# Autodesk Inventor assembly: Shooter Assembly
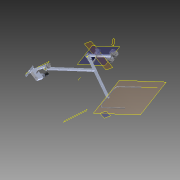
[picture p0: Inventor's stored thumbnail of the model, 180x180]
Saved by Autodesk Inventor 2014 (Build 180170000, 170)
## iProperties
Created: 2014-01-05
Part Number: Shooter Assembly
Document SubType Name: Assembly
Designer: Andrew Toennies
Mass: 1582.87 g
Surface Area: 6510.69 cm^2
Volume: 621.462 cm^3
Density: 2.54701 g/cm^3
Author: Andrew Toennies
## Documents named in this file (30)
- C:\Users\Andrew Toennies\Documents\GitHub\2014buildCAD\Shooter\Shooter Assembly.iam
- C:\Users\Andrew Toennies\Documents\GitHub\2014buildCAD\Shooter\Vex Pro 1x1 rectangular tubing 12 in length.ipt
- C:\Users\Andrew Toennies\Documents\GitHub\2014buildCAD\Shooter\Vex Pro End Bearing Mount.ipt
- C:\Users\Andrew Toennies\Documents\GitHub\2014buildCAD\Shooter\Vex Pro 1x1 rectangular tubing 27 in length.ipt
- C:\Users\Andrew Toennies\Documents\GitHub\2014buildCAD\Shooter\Vex Pro 1x1 rectangular tubing 24 in length.ipt
- C:\Users\Andrew Toennies\Documents\GitHub\2014buildCAD\Shooter\Vex Pro T gusset.ipt
- C:\Users\Andrew Toennies\Documents\GitHub\2014buildCAD\Shooter\Vex Pro Corner Gusset.ipt
- C:\Users\Andrew Toennies\Documents\GitHub\2014buildCAD\Shooter\Vex Pro 1x1 rectangular tubing 13 in length.ipt
- C:\Users\Andrew Toennies\Documents\GitHub\2014buildCAD\Shooter\Vex Pro Side Bearing Gusset.ipt
- C:\Users\Andrew Toennies\Documents\GitHub\2014buildCAD\Shooter\Bearing ID 0.500 Hex OD 1.125.ipt
- C:\Users\Andrew Toennies\Documents\GitHub\2014buildCAD\Shooter\Axle 0.500 Hex 5 in length.ipt
- C:\Users\Andrew Toennies\Documents\GitHub\2014buildCAD\Shooter\Spacer.ipt
- C:\Users\Andrew Toennies\Documents\GitHub\2014buildCAD\Shooter\Bearing ID 0.375 OD 1.125.ipt
- C:\Users\Andrew Toennies\Documents\GitHub\2014buildCAD\Shooter\Axle 0.375 3 in length.ipt
- C:\Users\Andrew Toennies\Documents\GitHub\2014buildCAD\Shooter\Vex Pro 30 tooth 9mm timing belt pulley.ipt
- C:\Users\Andrew Toennies\Documents\GitHub\2014buildCAD\Shooter\Vex Pro VersaHub 0.500 Hex.ipt
- C:\Users\Andrew Toennies\Documents\GitHub\2014buildCAD\Shooter\armbackspacer.ipt
- C:\Users\Andrew Toennies\Documents\GitHub\2014buildCAD\Shooter\Axle 0.500 Hex 3 in length.ipt
- C:\Users\Andrew Toennies\Documents\GitHub\2014buildCAD\Shooter\Worm-Drive-Gearbox-16to1.iam
- C:\Users\Andrew Toennies\Documents\GitHub\2014buildCAD\Shooter\Vex Pro 32 tooth 15 mm timing belt pulley.ipt
- C:\Users\Andrew Toennies\Documents\GitHub\2014buildCAD\Shooter\Vex Pro Traction 1 in wide 4 in dia wheel.iam
- C:\Users\Andrew Toennies\Documents\GitHub\2014buildCAD\Shooter\Aluminum Tube Bent 0.500 OD 0.436 ID.ipt
- C:\Users\Andrew Toennies\Documents\GitHub\2014buildCAD\Shooter\Bag Motor with VersaPlanetary 10 to 1 Reduction.iam
- C:\Users\Andrew Toennies\Documents\GitHub\2014buildCAD\Shooter\Vex Pro 18 tooth timing belt pulley.ipt
- C:\Users\Andrew Toennies\Documents\GitHub\2014buildCAD\Shooter\Vex Pro VersaPlanetary Face Mount.ipt
- C:\Users\Andrew Toennies\Documents\GitHub\2014buildCAD\Shooter\Pneumatic Cylinder Retracted (McMaster Part #6498K602).ipt
- C:\Users\Andrew Toennies\Documents\GitHub\2014buildCAD\Shooter\Foot Bracket Mount (McMaster Part #6498K710).ipt
- C:\Users\Andrew Toennies\Documents\GitHub\2014buildCAD\Shooter\Rod End (McMaster Part #6498K592).ipt
- C:\Users\Andrew Toennies\Documents\GitHub\2014buildCAD\Shooter\Spacer2.ipt
- C:\Users\Andrew Toennies\Documents\GitHub\2014buildCAD\Shooter\Bracket.ipt
## Components (46 placed, 29 different names)
1. Vex Pro 1x1 rectangular tubing 12 in length:1 — Flush:1, Insert:9, Insert:10, Insert:11, Insert:12, Flush:4, Mate:23, Mate:24, Mate:25, Mate:26, Mate:27, Mate:28, Mate:43, Mate:49, Mate:50, Angle:1
2. Vex Pro 1x1 rectangular tubing 27 in length:1 — Flush:1, Insert:5, Insert:6, Insert:7, Insert:8, Flush:2, Mate:2, Mate:33, Mate:34
3. Vex Pro 1x1 rectangular tubing 24 in length:1 — Flush:2, Mate:2, Flush:3, Mate:6, Flush:9, Mate:53, Mate:54, Angle:1, Flush:17, Angle:2, Flush:22, Flush:23, Mate:64, Mate:65, Flush:24, Insert:57, Insert:58
4. Vex Pro T gusset:1 — Insert:5, Insert:6, Mate:6
5. Vex Pro T gusset:2 — Insert:7, Insert:8
6. Vex Pro Corner Gusset:1 — Insert:9, Insert:10, Flush:6
7. Vex Pro Corner Gusset:2 — Insert:11, Insert:12
8. Vex Pro End Bearing Mount:3 — Insert:35, Insert:47, Insert:48, Angle:3
9. Vex Pro End Bearing Mount:4 — Insert:36, Insert:49, Insert:50
10. Vex Pro 1x1 rectangular tubing 13 in length:1 — Flush:3, Insert:21, Insert:22, Insert:23, Insert:24, Flush:8, Mate:51, Angle:2, Flush:19, Flush:20, Flush:21, Mate:63, Flush:25, Tangent:1, Insert:59, Insert:60, Insert:61, Insert:62
11. Vex Pro End Bearing Mount:5 — Insert:21, Insert:22, Insert:25
12. Vex Pro End Bearing Mount:6 — Insert:23, Insert:24, Insert:26
13. Bearing ID 0.500 Hex OD 1.125:1 — Insert:26, Flush:7, Mate:7, Mate:8
14. Bearing ID 0.500 Hex OD 1.125:2 — Insert:25, Flush:7, Mate:10, Mate:16
15. Axle 0.500 Hex 5 in length:1 — Mate:7, Mate:8, Flush:8, Flush:10, Flush:11, Mate:14, Mate:15, Mate:18, Mate:19, Mate:21, Mate:22, Flush:12, Flush:16
16. Spacer:1 — Insert:47, Insert:48, Mate:65, Flush:24
17. Spacer:2 — Insert:49, Insert:50, Flush:22, Flush:23, Mate:64
18. Bearing ID 0.375 OD 1.125:1 — Insert:35, Mate:9
19. Bearing ID 0.375 OD 1.125:2 — Insert:36, Mate:66
20. Axle 0.375 3 in length:1 — Mate:9, Flush:9, Mate:13, Mate:51, Mate:66
21. Vex Pro 30 tooth 9mm timing belt pulley:1 — Mate:14, Mate:15, Mate:16, Flush:18
22. Vex Pro VersaHub 0.500 Hex:1 — Mate:17, Mate:18, Mate:19, Flush:16, Insert:51
23. Vex Pro VersaHub 0.500 Hex:2 — Mate:17
24. Vex Pro VersaHub 0.500 Hex:3 — Mate:20, Mate:21, Mate:22, Flush:12, Mate:52
25. Vex Pro VersaHub 0.500 Hex:4 — Mate:20, Mate:52, Insert:52
26. armbackspacer:1 — Mate:26, Mate:27, Mate:28, Mate:29, Mate:30, Mate:31
27. armbackspacer:2 — Mate:23, Mate:24, Mate:25, Mate:32, Flush:13, Flush:14
28. Vex Pro Side Bearing Gusset:1 — Mate:29, Mate:30, Mate:31, Mate:35, Mate:36
29. Vex Pro Side Bearing Gusset:2 — Mate:32, Flush:13, Flush:14, Mate:37, Mate:38
30. Bearing ID 0.500 Hex OD 1.125:3 — Mate:35, Mate:36
31. Axle 0.500 Hex 3 in length:1 — Mate:33, Mate:34, Mate:39, Mate:40, Flush:15, Mate:47, Mate:48
32. Bearing ID 0.500 Hex OD 1.125:4 — Mate:37, Mate:38, Mate:39, Mate:40, Flush:15
33. Worm-Drive-Gearbox-16to1:1 [sub-assembly] — Mate:43, Mate:49, Mate:50
34. Vex Pro 32 tooth 15 mm timing belt pulley:1 — Mate:47, Mate:48
35. Vex Pro Traction 1 in wide 4 in dia wheel:1 [sub-assembly] — Insert:51
36. Vex Pro Traction 1 in wide 4 in dia wheel:2 [sub-assembly] — Insert:52
37. Aluminum Tube Bent 0.500 OD 0.436 ID:1 — Mate:53, Mate:54, Flush:17, Mate:67, Mate:68
38. Bag Motor with VersaPlanetary 10 to 1 Reduction:1 [sub-assembly] — Mate:55, Mate:56, Flush:19, Insert:53, Insert:54
39. Vex Pro 18 tooth timing belt pulley:1 — Mate:55, Mate:56, Flush:18
40. Vex Pro VersaPlanetary Face Mount:1 — Insert:53, Insert:54, Flush:21, Mate:63, Mate:75
41. Pneumatic Cylinder Retracted (McMaster Part #6498K602):1 — Insert:55, Insert:56
42. Foot Bracket Mount (McMaster Part #6498K710):1 — Insert:55, Mate:71, Mate:72, Mate:73
43. Rod End (McMaster Part #6498K592):1 — Insert:56, Mate:74, Tangent:1
44. Spacer2:1 — Insert:57, Insert:58, Mate:71, Mate:72, Mate:73
45. Bracket:1 — Insert:59, Insert:60
46. Bracket:2 — Insert:61, Insert:62
## Relationships (124: Mate 63, Insert 32, Flush 25, Angle 3, Tangent 1)
- Flush:1: Vex Pro 1x1 rectangular tubing 12 in length:1 ↔ Vex Pro 1x1 rectangular tubing 27 in length:1
- Insert:5: Vex Pro 1x1 rectangular tubing 27 in length:1 ↔ Vex Pro T gusset:1
- Insert:6: Vex Pro 1x1 rectangular tubing 27 in length:1 ↔ Vex Pro T gusset:1
- Insert:7: Vex Pro 1x1 rectangular tubing 27 in length:1 ↔ Vex Pro T gusset:2
- Insert:8: Vex Pro 1x1 rectangular tubing 27 in length:1 ↔ Vex Pro T gusset:2
- Flush:2: Vex Pro 1x1 rectangular tubing 27 in length:1 ↔ Vex Pro 1x1 rectangular tubing 24 in length:1
- Mate:2: Vex Pro 1x1 rectangular tubing 27 in length:1 ↔ Vex Pro 1x1 rectangular tubing 24 in length:1
- Insert:9: Vex Pro 1x1 rectangular tubing 12 in length:1 ↔ Vex Pro Corner Gusset:1
- Insert:10: Vex Pro 1x1 rectangular tubing 12 in length:1 ↔ Vex Pro Corner Gusset:1
- Insert:11: Vex Pro 1x1 rectangular tubing 12 in length:1 ↔ Vex Pro Corner Gusset:2
- Insert:12: Vex Pro 1x1 rectangular tubing 12 in length:1 ↔ Vex Pro Corner Gusset:2
- Flush:3: Vex Pro 1x1 rectangular tubing 24 in length:1 ↔ Vex Pro 1x1 rectangular tubing 13 in length:1
- Flush:4: Vex Pro 1x1 rectangular tubing 12 in length:1
- Mate:6: Vex Pro 1x1 rectangular tubing 24 in length:1 ↔ Vex Pro T gusset:1
- Flush:5 (-711.2 mm)
- Flush:6 (-1422.4 mm): Vex Pro Corner Gusset:1
- Insert:21: Vex Pro 1x1 rectangular tubing 13 in length:1 ↔ Vex Pro End Bearing Mount:5
- Insert:22: Vex Pro 1x1 rectangular tubing 13 in length:1 ↔ Vex Pro End Bearing Mount:5
- Insert:23: Vex Pro 1x1 rectangular tubing 13 in length:1 ↔ Vex Pro End Bearing Mount:6
- Insert:24: Vex Pro 1x1 rectangular tubing 13 in length:1 ↔ Vex Pro End Bearing Mount:6
- Insert:25: Vex Pro End Bearing Mount:5 ↔ Bearing ID 0.500 Hex OD 1.125:2
- Insert:26: Vex Pro End Bearing Mount:6 ↔ Bearing ID 0.500 Hex OD 1.125:1
- Flush:7: Bearing ID 0.500 Hex OD 1.125:1 ↔ Bearing ID 0.500 Hex OD 1.125:2
- Mate:7: Bearing ID 0.500 Hex OD 1.125:1 ↔ Axle 0.500 Hex 5 in length:1
- Mate:8: Bearing ID 0.500 Hex OD 1.125:1 ↔ Axle 0.500 Hex 5 in length:1
- Flush:8 (-63.5 mm): Vex Pro 1x1 rectangular tubing 13 in length:1 ↔ Axle 0.500 Hex 5 in length:1
- Insert:35: Vex Pro End Bearing Mount:3 ↔ Bearing ID 0.375 OD 1.125:1
- Insert:36: Vex Pro End Bearing Mount:4 ↔ Bearing ID 0.375 OD 1.125:2
- Mate:9: Bearing ID 0.375 OD 1.125:1 ↔ Axle 0.375 3 in length:1
- Flush:9 (-25.4 mm): Vex Pro 1x1 rectangular tubing 24 in length:1 ↔ Axle 0.375 3 in length:1
- Mate:10: Bearing ID 0.500 Hex OD 1.125:2
- Flush:10 (-4.7625 mm): Axle 0.500 Hex 5 in length:1
- Flush:11 (-4.7625 mm): Axle 0.500 Hex 5 in length:1
- Mate:11
- Mate:12
- Mate:13: Axle 0.375 3 in length:1
- Mate:14: Axle 0.500 Hex 5 in length:1 ↔ Vex Pro 30 tooth 9mm timing belt pulley:1
- Mate:15: Axle 0.500 Hex 5 in length:1 ↔ Vex Pro 30 tooth 9mm timing belt pulley:1
- Mate:16: Bearing ID 0.500 Hex OD 1.125:2 ↔ Vex Pro 30 tooth 9mm timing belt pulley:1
- Mate:17: Vex Pro VersaHub 0.500 Hex:1 ↔ Vex Pro VersaHub 0.500 Hex:2
- Mate:18: Axle 0.500 Hex 5 in length:1 ↔ Vex Pro VersaHub 0.500 Hex:1
- Mate:19: Axle 0.500 Hex 5 in length:1 ↔ Vex Pro VersaHub 0.500 Hex:1
- Mate:20: Vex Pro VersaHub 0.500 Hex:3 ↔ Vex Pro VersaHub 0.500 Hex:4
- Mate:21: Axle 0.500 Hex 5 in length:1 ↔ Vex Pro VersaHub 0.500 Hex:3
- Mate:22: Axle 0.500 Hex 5 in length:1 ↔ Vex Pro VersaHub 0.500 Hex:3
- Flush:12 (9.525 mm): Axle 0.500 Hex 5 in length:1 ↔ Vex Pro VersaHub 0.500 Hex:3
- Mate:23: Vex Pro 1x1 rectangular tubing 12 in length:1 ↔ armbackspacer:2
- Mate:24: Vex Pro 1x1 rectangular tubing 12 in length:1 ↔ armbackspacer:2
- Mate:25: Vex Pro 1x1 rectangular tubing 12 in length:1 ↔ armbackspacer:2
- Mate:26: Vex Pro 1x1 rectangular tubing 12 in length:1 ↔ armbackspacer:1
- Mate:27: Vex Pro 1x1 rectangular tubing 12 in length:1 ↔ armbackspacer:1
- Mate:28: Vex Pro 1x1 rectangular tubing 12 in length:1 ↔ armbackspacer:1
- Mate:29: armbackspacer:1 ↔ Vex Pro Side Bearing Gusset:1
- Mate:30: armbackspacer:1 ↔ Vex Pro Side Bearing Gusset:1
- Mate:31: armbackspacer:1 ↔ Vex Pro Side Bearing Gusset:1
- Mate:32: armbackspacer:2 ↔ Vex Pro Side Bearing Gusset:2
- Flush:13: armbackspacer:2 ↔ Vex Pro Side Bearing Gusset:2
- Flush:14: armbackspacer:2 ↔ Vex Pro Side Bearing Gusset:2
- Mate:33: Vex Pro 1x1 rectangular tubing 27 in length:1 ↔ Axle 0.500 Hex 3 in length:1
- Mate:34: Vex Pro 1x1 rectangular tubing 27 in length:1 ↔ Axle 0.500 Hex 3 in length:1
- Mate:35: Vex Pro Side Bearing Gusset:1 ↔ Bearing ID 0.500 Hex OD 1.125:3
- Mate:36: Vex Pro Side Bearing Gusset:1 ↔ Bearing ID 0.500 Hex OD 1.125:3
- Mate:37: Vex Pro Side Bearing Gusset:2 ↔ Bearing ID 0.500 Hex OD 1.125:4
- Mate:38: Vex Pro Side Bearing Gusset:2 ↔ Bearing ID 0.500 Hex OD 1.125:4
- Mate:39: Axle 0.500 Hex 3 in length:1 ↔ Bearing ID 0.500 Hex OD 1.125:4
- Mate:40: Axle 0.500 Hex 3 in length:1 ↔ Bearing ID 0.500 Hex OD 1.125:4
- Flush:15 (-9.525 mm): Axle 0.500 Hex 3 in length:1 ↔ Bearing ID 0.500 Hex OD 1.125:4
- Flush:16 (12.7 mm): Axle 0.500 Hex 5 in length:1 ↔ Vex Pro VersaHub 0.500 Hex:1
- Mate:43: Vex Pro 1x1 rectangular tubing 12 in length:1 ↔ Worm-Drive-Gearbox-16to1:1
- Mate:47: Axle 0.500 Hex 3 in length:1 ↔ Vex Pro 32 tooth 15 mm timing belt pulley:1
- Mate:48: Axle 0.500 Hex 3 in length:1 ↔ Vex Pro 32 tooth 15 mm timing belt pulley:1
- Mate:49: Vex Pro 1x1 rectangular tubing 12 in length:1 ↔ Worm-Drive-Gearbox-16to1:1
- Mate:50: Vex Pro 1x1 rectangular tubing 12 in length:1 ↔ Worm-Drive-Gearbox-16to1:1
- Insert:47: Vex Pro End Bearing Mount:3 ↔ Spacer:1
- Insert:48: Vex Pro End Bearing Mount:3 ↔ Spacer:1
- Insert:49: Vex Pro End Bearing Mount:4 ↔ Spacer:2
- Insert:50: Vex Pro End Bearing Mount:4 ↔ Spacer:2
- Mate:51: Vex Pro 1x1 rectangular tubing 13 in length:1 ↔ Axle 0.375 3 in length:1
- Mate:52: Vex Pro VersaHub 0.500 Hex:3 ↔ Vex Pro VersaHub 0.500 Hex:4
- Insert:51: Vex Pro VersaHub 0.500 Hex:1 ↔ Vex Pro Traction 1 in wide 4 in dia wheel:1
- Insert:52: Vex Pro VersaHub 0.500 Hex:4 ↔ Vex Pro Traction 1 in wide 4 in dia wheel:2
- Mate:53: Vex Pro 1x1 rectangular tubing 24 in length:1 ↔ Aluminum Tube Bent 0.500 OD 0.436 ID:1
- Mate:54 (171.45 mm): Vex Pro 1x1 rectangular tubing 24 in length:1 ↔ Aluminum Tube Bent 0.500 OD 0.436 ID:1
- Angle:1 (90 deg): Vex Pro 1x1 rectangular tubing 12 in length:1 ↔ Vex Pro 1x1 rectangular tubing 24 in length:1
- Flush:17 (342.9 mm): Vex Pro 1x1 rectangular tubing 24 in length:1 ↔ Aluminum Tube Bent 0.500 OD 0.436 ID:1
- Angle:2 (270 deg): Vex Pro 1x1 rectangular tubing 24 in length:1 ↔ Vex Pro 1x1 rectangular tubing 13 in length:1
- Mate:55: Bag Motor with VersaPlanetary 10 to 1 Reduction:1 ↔ Vex Pro 18 tooth timing belt pulley:1
- Mate:56: Bag Motor with VersaPlanetary 10 to 1 Reduction:1 ↔ Vex Pro 18 tooth timing belt pulley:1
- Flush:18: Vex Pro 30 tooth 9mm timing belt pulley:1 ↔ Vex Pro 18 tooth timing belt pulley:1
- Flush:19: Vex Pro 1x1 rectangular tubing 13 in length:1 ↔ Bag Motor with VersaPlanetary 10 to 1 Reduction:1
- Mate:60
- Mate:61
- Flush:20 (-12.7 mm): Vex Pro 1x1 rectangular tubing 13 in length:1
- Mate:62
- Insert:53: Bag Motor with VersaPlanetary 10 to 1 Reduction:1 ↔ Vex Pro VersaPlanetary Face Mount:1
- Insert:54: Bag Motor with VersaPlanetary 10 to 1 Reduction:1 ↔ Vex Pro VersaPlanetary Face Mount:1
- Flush:21: Vex Pro 1x1 rectangular tubing 13 in length:1 ↔ Vex Pro VersaPlanetary Face Mount:1
- Mate:63: Vex Pro 1x1 rectangular tubing 13 in length:1 ↔ Vex Pro VersaPlanetary Face Mount:1
- Flush:22: Vex Pro 1x1 rectangular tubing 24 in length:1 ↔ Spacer:2
- Flush:23: Vex Pro 1x1 rectangular tubing 24 in length:1 ↔ Spacer:2
- Mate:64: Vex Pro 1x1 rectangular tubing 24 in length:1 ↔ Spacer:2
- Mate:65: Vex Pro 1x1 rectangular tubing 24 in length:1 ↔ Spacer:1
- Flush:24: Vex Pro 1x1 rectangular tubing 24 in length:1 ↔ Spacer:1
- Mate:66: Bearing ID 0.375 OD 1.125:2 ↔ Axle 0.375 3 in length:1
- Mate:67: Aluminum Tube Bent 0.500 OD 0.436 ID:1
- Mate:68: Aluminum Tube Bent 0.500 OD 0.436 ID:1
- Mate:69
- Mate:70
- Flush:25 (-12.7 mm): Vex Pro 1x1 rectangular tubing 13 in length:1
- Insert:55: Pneumatic Cylinder Retracted (McMaster Part #6498K602):1 ↔ Foot Bracket Mount (McMaster Part #6498K710):1
- Insert:56 (-12.7 mm): Pneumatic Cylinder Retracted (McMaster Part #6498K602):1 ↔ Rod End (McMaster Part #6498K592):1
- Insert:57: Vex Pro 1x1 rectangular tubing 24 in length:1 ↔ Spacer2:1
- Insert:58: Vex Pro 1x1 rectangular tubing 24 in length:1 ↔ Spacer2:1
- Mate:71: Foot Bracket Mount (McMaster Part #6498K710):1 ↔ Spacer2:1
- Mate:72: Foot Bracket Mount (McMaster Part #6498K710):1 ↔ Spacer2:1
- Mate:73: Foot Bracket Mount (McMaster Part #6498K710):1 ↔ Spacer2:1
- Mate:74: Rod End (McMaster Part #6498K592):1
- Angle:3 (0 deg): Vex Pro End Bearing Mount:3
- Tangent:1: Vex Pro 1x1 rectangular tubing 13 in length:1 ↔ Rod End (McMaster Part #6498K592):1
- Insert:59: Vex Pro 1x1 rectangular tubing 13 in length:1 ↔ Bracket:1
- Insert:60: Vex Pro 1x1 rectangular tubing 13 in length:1 ↔ Bracket:1
- Insert:61: Vex Pro 1x1 rectangular tubing 13 in length:1 ↔ Bracket:2
- Insert:62: Vex Pro 1x1 rectangular tubing 13 in length:1 ↔ Bracket:2
- Mate:75: Vex Pro VersaPlanetary Face Mount:1
